# Autodesk Inventor assembly: 000100
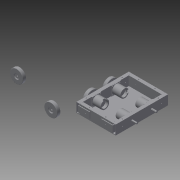
[picture p0: Inventor's stored thumbnail of the model, 180x180]
Saved by Autodesk Inventor 2015 (Build 190159000, 159)
## iProperties
Created: 2015-05-18
Part Number: 000100
Document SubType Name: Assembly
Designer: Wesley
Author: Wesley
## Documents named in this file (10)
- C:\Users\Wesley\Documents\GitHub\EngineeringFinal\Engineering\Engineering Documentation\CADS\0001__\000100.iam
- C:\Users\Wesley\Documents\GitHub\EngineeringFinal\Engineering\Engineering Documentation\CADS\0001__\000101-1.ipt
- C:\Users\Wesley\Documents\GitHub\EngineeringFinal\Engineering\Engineering Documentation\CADS\0001__\000101-2.ipt
- C:\Users\Wesley\Documents\GitHub\EngineeringFinal\Engineering\Engineering Documentation\CADS\0001__\000102.ipt
- C:\Users\Wesley\Documents\GitHub\EngineeringFinal\Engineering\Engineering Documentation\CADS\0001__\000103.ipt
- C:\Users\Wesley\Documents\GitHub\EngineeringFinal\Engineering\Engineering Documentation\CADS\0001__\000104.ipt
- C:\Users\Wesley\Documents\GitHub\EngineeringFinal\Engineering\Engineering Documentation\CADS\0001__\000111.ipt
- C:\Users\Wesley\Documents\GitHub\EngineeringFinal\Engineering\Engineering Documentation\CADS\0001__\000109.ipt
- C:\Users\Wesley\Documents\GitHub\EngineeringFinal\Engineering\Engineering Documentation\CADS\0001__\000108-1.ipt
- C:\Users\Wesley\Documents\GitHub\EngineeringFinal\Engineering\Engineering Documentation\CADS\0001__\000110.ipt
## Components (27 placed, 9 different names)
1. 000101-1:1 — Mate:1, Flush:1, Flush:2, Flush:6, Mate:3, Mate:5, Mate:10, Mate:12, Mate:16, Flush:9, Mate:17, Mate:23, Mate:34, Mate:36, Mate:38, Mate:40
2. 000101-2:1 — Mate:1, Flush:1, Flush:2, Mate:2, Flush:3, Flush:4, Mate:4, Mate:6, Mate:7, Mate:11
3. 000101-1:2 — Mate:2, Flush:3, Flush:4, Flush:7, Mate:8, Mate:14, Mate:18, Mate:47, Mate:48, Mate:52, Mate:53
4. 000101-2:2 — Flush:6, Mate:3, Flush:7, Mate:9, Mate:13, Mate:15, Flush:8
5. 000102:1 — Mate:4, Mate:5, Mate:6
6. 000102:2 — Mate:9, Mate:10, Mate:12
7. 000102:3 — Mate:7, Mate:8, Mate:11
8. 000102:4 — Mate:13, Mate:14, Mate:15
9. 000103:1 — Mate:16, Flush:8, Flush:9, Mate:17, Mate:18, Mate:35, Mate:37, Mate:49, Mate:54
10. 000104:1
11. 000104:2 — Mate:39, Mate:40, Mate:41, Mate:42
12. 000104:3 — Mate:19, Mate:26, Mate:27
13. 000104:4
14. 000111:1 — Mate:19, Mate:21, Mate:22
15. 000109:1 — Mate:21, Mate:22, Mate:23, Mate:32, Mate:33
16. 000108-1:1 — Mate:26, Mate:27
17. 000109:2 — Mate:43, Mate:44, Mate:46
18. 000109:3 — Mate:28, Mate:29, Mate:30, Mate:31
19. 000109:4 — Mate:50, Mate:51, Mate:56
20. 000111:2 — Mate:55, Mate:56
21. 000111:3 — Mate:45, Mate:46
22. 000111:4 — Mate:28, Mate:29
23. 000110:1 — Mate:30, Mate:31, Mate:36, Mate:37, Mate:38, Mate:39
24. 000110:2 — Mate:32, Mate:33, Mate:34, Mate:35
25. 000108-1:2 — Mate:41, Mate:42
26. 000110:3 — Mate:43, Mate:44, Mate:45, Mate:47, Mate:48, Mate:49
27. 000110:4 — Mate:50, Mate:51, Mate:52, Mate:53, Mate:54, Mate:55
## Relationships (61: Mate 53, Flush 8)
- Mate:1: 000101-1:1 ↔ 000101-2:1
- Flush:1: 000101-1:1 ↔ 000101-2:1
- Flush:2: 000101-1:1 ↔ 000101-2:1
- Mate:2: 000101-2:1 ↔ 000101-1:2
- Flush:3: 000101-2:1 ↔ 000101-1:2
- Flush:4: 000101-2:1 ↔ 000101-1:2
- Flush:6: 000101-1:1 ↔ 000101-2:2
- Mate:3: 000101-1:1 ↔ 000101-2:2
- Flush:7: 000101-1:2 ↔ 000101-2:2
- Mate:4: 000101-2:1 ↔ 000102:1
- Mate:5: 000101-1:1 ↔ 000102:1
- Mate:6: 000101-2:1 ↔ 000102:1
- Mate:7: 000101-2:1 ↔ 000102:3
- Mate:8: 000101-1:2 ↔ 000102:3
- Mate:9: 000101-2:2 ↔ 000102:2
- Mate:10: 000101-1:1 ↔ 000102:2
- Mate:11: 000101-2:1 ↔ 000102:3
- Mate:12: 000101-1:1 ↔ 000102:2
- Mate:13: 000101-2:2 ↔ 000102:4
- Mate:14: 000101-1:2 ↔ 000102:4
- Mate:15: 000101-2:2 ↔ 000102:4
- Mate:16: 000101-1:1 ↔ 000103:1
- Flush:8: 000101-2:2 ↔ 000103:1
- Flush:9: 000101-1:1 ↔ 000103:1
- Mate:17: 000101-1:1 ↔ 000103:1
- Mate:18: 000101-1:2 ↔ 000103:1
- Mate:19: 000104:3 ↔ 000111:1
- Mate:21: 000111:1 ↔ 000109:1
- Mate:22: 000111:1 ↔ 000109:1
- Mate:23: 000101-1:1 ↔ 000109:1
- Mate:26: 000104:3 ↔ 000108-1:1
- Mate:27: 000104:3 ↔ 000108-1:1
- Mate:28: 000109:3 ↔ 000111:4
- Mate:29: 000109:3 ↔ 000111:4
- Mate:30: 000109:3 ↔ 000110:1
- Mate:31: 000109:3 ↔ 000110:1
- Mate:32: 000109:1 ↔ 000110:2
- Mate:33: 000109:1 ↔ 000110:2
- Mate:34: 000101-1:1 ↔ 000110:2
- Mate:35: 000103:1 ↔ 000110:2
- Mate:36: 000101-1:1 ↔ 000110:1
- Mate:37: 000103:1 ↔ 000110:1
- Mate:38: 000101-1:1 ↔ 000110:1
- Mate:39: 000104:2 ↔ 000110:1
- Mate:40 (1.27 mm): 000101-1:1 ↔ 000104:2
- Mate:41: 000104:2 ↔ 000108-1:2
- Mate:42: 000104:2 ↔ 000108-1:2
- Mate:43: 000109:2 ↔ 000110:3
- Mate:44: 000109:2 ↔ 000110:3
- Mate:45: 000111:3 ↔ 000110:3
- Mate:46: 000109:2 ↔ 000111:3
- Mate:47: 000101-1:2 ↔ 000110:3
- Mate:48: 000101-1:2 ↔ 000110:3
- Mate:49: 000103:1 ↔ 000110:3
- Mate:50: 000109:4 ↔ 000110:4
- Mate:51: 000109:4 ↔ 000110:4
- Mate:52: 000101-1:2 ↔ 000110:4
- Mate:53: 000101-1:2 ↔ 000110:4
- Mate:54: 000103:1 ↔ 000110:4
- Mate:55: 000111:2 ↔ 000110:4
- Mate:56: 000109:4 ↔ 000111:2
